# Autodesk Inventor assembly: cabinet
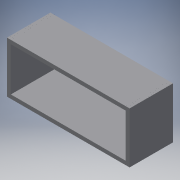
[picture p0: Inventor's stored thumbnail of the model, 180x180]
Saved by Autodesk Inventor 2016 (Build 200138000, 138)
## iProperties
Created: 2015-10-24
Part Number: cabinet
Document SubType Name: Assembly
Designer: jeremyhale
Author: jeremyhale
## Documents named in this file (4)
- \\psf\Home\Documents\Poorhouse\git\p0001\cabinet.iam
- \\psf\Home\Documents\Poorhouse\git\p0001\cabinet-bottom.ipt
- \\psf\Home\Documents\Poorhouse\git\p0001\cabinet-side.ipt
- \\psf\Home\Documents\Poorhouse\git\p0001\cabinet-top.ipt
## Components (4 placed, 3 different names)
1. bottom — Flush:3, Flush:4, Rigid:1
2. top — Rigid:2
3. cabinet-side:1 — Flush:5, Rigid:1, Rigid:2
4. cabinet-side:2
## Component patterns: sides (2 elements)
## Relationships (5: Flush 3, WeldJoint 2)
- Flush:3: bottom
- Flush:4: bottom
- Flush:5: cabinet-side:1
- Rigid:1 [WeldJoint]: bottom ↔ cabinet-side:1
- Rigid:2 [WeldJoint]: top ↔ cabinet-side:1
